# Autodesk Inventor assembly: Elevator Motor Assembly_MIR1 (nano) attempt
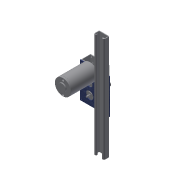
[picture p0: Inventor's stored thumbnail of the model, 180x180]
Saved by Autodesk Inventor 2015 (Build 190159000, 159)
## iProperties
Created: 2015-01-24
Part Number: Elevator Motor Assembly_MIR1 (nano) attempt
Document SubType Name: Assembly
Designer: Peter
Author: Peter
## Documents named in this file (4)
- C:\Users\Noah\Desktop\Alternate Parts for Nano Toughbox\Elevator Motor Assembly_MIR1 (nano) attempt.iam
- C:\Users\Noah\Desktop\Alternate Parts for Nano Toughbox\Andy Mark Tough Box Nano.iam
- C:\Users\Noah\Desktop\Alternate Parts for Nano Toughbox\c channel for mounting plate 760 first hole.ipt
- C:\Users\Noah\Desktop\Alternate Parts for Nano Toughbox\attatching plate for toughbox.ipt
## Components (3 placed, 3 different names)
1. Andy Mark Tough Box Nano:1 [sub-assembly] — Mate:1, Mate:2, Flush:1, Mate:4, Flush:5
2. c channel for mounting plate 760 first hole:1 — Mate:1, Mate:2, Flush:1, Flush:4
3. attatching plate for toughbox:1 — Flush:4, Mate:4, Flush:5
## Relationships (6: Mate 3, Flush 3)
- Mate:1 (2.286 mm): Andy Mark Tough Box Nano:1 ↔ c channel for mounting plate 760 first hole:1
- Mate:2: Andy Mark Tough Box Nano:1 ↔ c channel for mounting plate 760 first hole:1
- Flush:1 (139.1158 mm): Andy Mark Tough Box Nano:1 ↔ c channel for mounting plate 760 first hole:1
- Flush:4: c channel for mounting plate 760 first hole:1 ↔ attatching plate for toughbox:1
- Mate:4: Andy Mark Tough Box Nano:1 ↔ attatching plate for toughbox:1
- Flush:5: Andy Mark Tough Box Nano:1 ↔ attatching plate for toughbox:1
